# Autodesk Inventor assembly: ANDGATEASSEMBLY
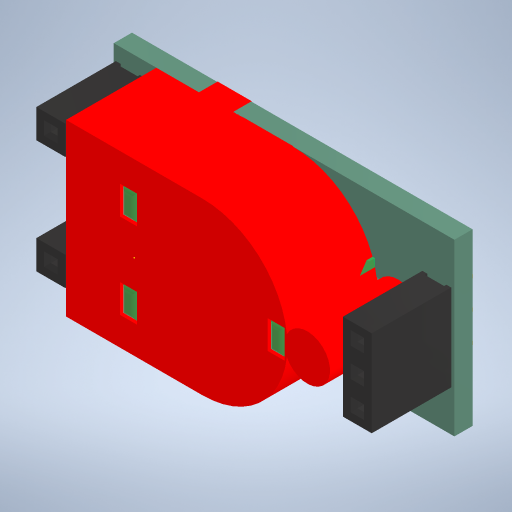
[picture p0: Inventor's stored thumbnail of the model, 512x512]
Saved by Autodesk Inventor 2024 (Build 280153000, 153)
## iProperties
Created: 2024-01-22
Part Number: ANDGATEASSEMBLY
Document SubType Name: Assembly
Designer: Jetsan
Author: Jetsan
## Documents named in this file (4)
- C:\Git\Personal\DigitalLogicProject\Models\ANDGATE\ANDGATEASSEMBLY.iam
- C:\Git\Personal\DigitalLogicProject\Models\LIGHTPIPING\LightPipe.ipt
- C:\Git\Personal\DigitalLogicProject\PCBS\GATE\GATE PCB.ipt
- C:\Git\Personal\DigitalLogicProject\Models\NANDGATE\NANDGATE.ipt
## Components (5 placed, 3 different names)
1. LightPipe:1 — Mate:3, Mate:6, Mate:7
2. LightPipe:2 — Mate:4, Mate:8, Mate:9
3. NANDGATE:1 — Flush:1, Mate:5, Mate:6, Mate:7, Mate:8, Mate:9, Mate:11, Mate:12
4. GATE PCB:1 — Mate:3, Mate:4, Flush:1, Mate:5, Mate:10
5. LightPipe:3 — Mate:10, Mate:11, Mate:12
## Relationships (11: Mate 10, Flush 1)
- Mate:3: LightPipe:1 ↔ GATE PCB:1
- Mate:4: LightPipe:2 ↔ GATE PCB:1
- Flush:1: NANDGATE:1 ↔ GATE PCB:1
- Mate:5: NANDGATE:1 ↔ GATE PCB:1
- Mate:6: LightPipe:1 ↔ NANDGATE:1
- Mate:7: LightPipe:1 ↔ NANDGATE:1
- Mate:8: LightPipe:2 ↔ NANDGATE:1
- Mate:9: LightPipe:2 ↔ NANDGATE:1
- Mate:10: GATE PCB:1 ↔ LightPipe:3
- Mate:11: NANDGATE:1 ↔ LightPipe:3
- Mate:12: NANDGATE:1 ↔ LightPipe:3
